# Autodesk Inventor assembly: 4150RobotComplete v3 11.18.14
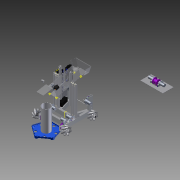
[picture p0: Inventor's stored thumbnail of the model, 180x180]
Saved by Autodesk Inventor 2015 SP1 (Build 190203100, 203)
## iProperties
Created: 2014-09-14
Part Number: 4150RobotComplete v3 11.18.14
Document SubType Name: Assembly
Designer: Family Room
Author: Family Room
## Documents named in this file (35)
- C:\Users\sapatel\Documents\GitHub\CAD\2014_robotComplete\4150RobotComplete v3 11.18.14.iam
- C:\Users\sapatel\Documents\GitHub\CAD\2014_robotComplete\Frame Side.ipt
- C:\Users\sapatel\Documents\GitHub\CAD\2014_robotComplete\center brace.ipt
- C:\Users\sapatel\Documents\GitHub\CAD\2014_robotComplete\Goal Guide 2.ipt
- C:\Users\sapatel\Documents\GitHub\CAD\2014_robotComplete\Hex bearing.ipt
- C:\Users\sapatel\Documents\GitHub\CAD\2014_robotComplete\Axle.ipt
- C:\Users\sapatel\Documents\GitHub\CAD\2014_robotComplete\Hex Collar.ipt
- C:\Users\sapatel\Documents\GitHub\CAD\2014_robotComplete\Hex Sprocket.ipt
- C:\Users\sapatel\Documents\GitHub\CAD\2014_robotComplete\left mecanum.iam
- C:\Users\sapatel\Documents\GitHub\CAD\2014_robotComplete\right mecanum.iam
- C:\Users\sapatel\Documents\GitHub\CAD\2014_robotComplete\Imported Components\motor mount\motor mount.ipt
- C:\Users\sapatel\Documents\GitHub\CAD\2014_robotComplete\Imported Components\motor\motor.iam
- C:\Users\sapatel\Documents\GitHub\CAD\2014_robotComplete\Imported Components\16t Sprocket\16t Sprocket.ipt
- C:\Users\sapatel\Documents\GitHub\CAD\2014_robotComplete\Imported Components\Motor Hub\Motor Hub.ipt
- C:\Users\sapatel\Documents\GitHub\CAD\2014_robotComplete\ball shoot.ipt
- C:\Users\sapatel\Documents\GitHub\CAD\2014_robotComplete\Imported Components\gusset\gusset.ipt
- C:\Users\sapatel\Documents\GitHub\CAD\2014_robotComplete\Lift Section.ipt
- C:\Users\sapatel\Documents\GitHub\CAD\2014_robotComplete\Lift Slider.ipt
- C:\Users\sapatel\Documents\GitHub\CAD\2014_robotComplete\Ball Collection Mechanism.iam
- C:\Users\sapatel\Documents\GitHub\CAD\2014_robotComplete\Bushing .ipt
- C:\Users\sapatel\Documents\GitHub\CAD\2014_robotComplete\BallShoot Axle.ipt
- C:\Users\sapatel\Documents\GitHub\CAD\2014_robotComplete\Rolling_Goal-30cm.iam
- C:\Users\sapatel\Documents\GitHub\CAD\2014_robotComplete\Spinner brace.ipt
- C:\Users\sapatel\Documents\GitHub\CAD\2014_robotComplete\Bushing 1.ipt
- C:\Users\sapatel\Documents\GitHub\CAD\2014_robotComplete\Imported Components\tetrix axle\tetrix axle.ipt
- C:\Users\sapatel\Documents\GitHub\CAD\winch assembly.iam
- C:\Users\sapatel\Documents\GitHub\CAD\2014_robotComplete\Winch baseplate.ipt
- C:\Users\sapatel\Documents\GitHub\CAD\2014_robotComplete\plate 1.ipt
- C:\Users\sapatel\Documents\GitHub\CAD\COTSParts\Tetrix\NXT brick.ipt
- C:\Users\sapatel\Documents\GitHub\CAD\COTSParts\Tetrix\NXT battery cover.ipt
- C:\Users\sapatel\Documents\GitHub\CAD\COTSParts\Tetrix\Tetrix Battery.ipt
- C:\Users\sapatel\Documents\GitHub\CAD\COTSParts\Tetrix\Tetrix DC motor controller.ipt
- C:\Users\sapatel\Documents\GitHub\CAD\COTSParts\Tetrix\Tetrix servo controller.ipt
- C:\Users\sapatel\Documents\GitHub\CAD\COTSParts\Tetrix\Tetrix power switch.ipt
- C:\Users\sapatel\Documents\GitHub\CAD\Electrical\samantha.ipt
## Components (100 placed, 34 different names)
1. Frame Side:2 — Flush:3, Flush:4, Mate:5, Flush:17, Mate:6, Flush:18, Flush:23, Flush:24, Mate:13, Flush:25, Insert:3, Insert:4, Flush:29, Flush:30, Flush:33, Mate:67, Mate:70, Mate:71, Flush:70, Mate:134, Flush:91, Mate:138, Mate:144, Flush:98, Mate:146, Flush:100, Flush:101
2. Frame Side:3 — Flush:3, Flush:4, Mate:7, Mate:15, Flush:26, Insert:1, Insert:2, Flush:27, Flush:28, Mate:63, Flush:31, Mate:65, Mate:72, Flush:71, Mate:132, Mate:142, Flush:97, Mate:147, Flush:102, Flush:103
3. center brace:1 — Mate:6, Flush:18, Mate:7, Flush:24, Mate:14, Mate:16, Angle:2, Angle:3
4. center brace:2 — Mate:5, Flush:17, Flush:23, Mate:90, Mate:117, Flush:96, Mate:143, Mate:145, Flush:99, Flush:107
5. Goal Guide 2:1 — Mate:13, Flush:25, Mate:14
6. Goal Guide 2:2 — Mate:15, Flush:26, Mate:16
7. Hex bearing:1 — Insert:1, Mate:17, Mate:28, Mate:35
8. Hex bearing:2 — Insert:2, Mate:18, Mate:22, Mate:36
9. Hex bearing:3 — Insert:4, Mate:19, Mate:24, Mate:37
10. Hex bearing:4 — Insert:3, Mate:20, Mate:30, Mate:38
11. Axle:1 — Mate:17, Flush:27, Mate:27, Mate:34, Mate:41, Mate:51, Mate:55
12. Axle:2 — Mate:18, Flush:28, Mate:21, Mate:33, Mate:42, Mate:52, Mate:56
13. Axle:3 — Mate:19, Flush:29, Mate:23, Mate:32, Mate:39, Mate:44
14. Axle:4 — Mate:20, Flush:30, Mate:29, Mate:31, Mate:40, Mate:43, Mate:57
15. Hex Collar:1 — Mate:21, Mate:22
16. Hex Collar:2 — Mate:23, Mate:24
17. Hex Collar:3 — Mate:29, Mate:30
18. Hex Collar:4 — Mate:27, Mate:28
19. Hex Sprocket:1 — Mate:31, Mate:38, Mate:46, Flush:41
20. Hex Sprocket:2 — Mate:32, Mate:37, Mate:45
21. Hex Sprocket:3 — Mate:34, Mate:35, Mate:48
22. Hex Sprocket:4 — Mate:33, Mate:36, Mate:47, Flush:39
23. left mecanum:1 [sub-assembly] — Mate:40, Mate:49, Mate:59
24. left mecanum:2 [sub-assembly] — Mate:39, Mate:50, Mate:58, Mate:60
25. Hex Collar:5 — Mate:43, Mate:46, Mate:49
26. Hex Collar:6 — Mate:41, Mate:48, Mate:53
27. Hex Collar:7 — Mate:42, Mate:47, Mate:54
28. Hex Collar:8 — Mate:44, Mate:45, Mate:50
29. right mecanum:1 [sub-assembly] — Mate:52, Mate:54, Mate:61
30. right mecanum:2 [sub-assembly] — Mate:51, Mate:53, Mate:62
31. Hex Collar:9 — Mate:57, Mate:59
32. Hex Collar:10 — Mate:58, Mate:60
33. Hex Collar:11 — Mate:55, Mate:62
34. Hex Collar:12 — Mate:56, Mate:61
35. motor mount:1 — Mate:69, Flush:34, Mate:70, Mate:75, Flush:38
36. motor mount:2 — Flush:33, Mate:67, Mate:69, Flush:34, Mate:71, Mate:76, Flush:37
37. motor mount:3 — Mate:63, Flush:31, Mate:66, Flush:32, Mate:72, Mate:73, Flush:35
38. motor mount:4 — Mate:65, Mate:66, Flush:32, Mate:74, Flush:36
39. motor:1 [sub-assembly] — Mate:73, Flush:35, Mate:80
40. motor:2 [sub-assembly] — Mate:74, Flush:36, Mate:81
41. motor:3 [sub-assembly] — Mate:76, Flush:37, Mate:77
42. motor:4 [sub-assembly] — Mate:75, Flush:38, Mate:78
43. 16t Sprocket:1 — Insert:8, Mate:78, Flush:42
44. 16t Sprocket:2 — Insert:7, Mate:77, Flush:41, Flush:42
45. 16t Sprocket:3 — Insert:9, Flush:39, Flush:40
46. 16t Sprocket:4 — Insert:5, Mate:80, Flush:40
47. Motor Hub:1 — Insert:8
48. Motor Hub:2 — Insert:7
49. Motor Hub:3 — Mate:81, Insert:9
50. Motor Hub:4 — Insert:5
51. ball shoot:1 — Mate:142, Flush:97, Mate:143
52. ball shoot:2 — Mate:144, Flush:98, Mate:145, Mate:158
53. Lift Section:1 — Mate:92, Flush:51, Flush:52, Mate:98, Flush:57, Flush:58, Flush:93, Flush:95, Insert:11
54. Lift Section:2 — Mate:90, Mate:117, Flush:71, Mate:123, Flush:82, Mate:124, Flush:83, Mate:125, Flush:84, Mate:131, Mate:133
55. Lift Slider:1 — Mate:92, Flush:51, Flush:52, Mate:103
56. Lift Slider:3 — Mate:95, Flush:54, Flush:55, Mate:100, Mate:102
57. Lift Slider:4 — Mate:96, Mate:97, Flush:56, Mate:98, Mate:103
58. Lift Section:3 — Mate:95, Flush:54, Flush:55, Flush:59, Flush:60, Mate:111, Flush:66, Mate:112, Flush:69, Angle:1
59. Lift Section:4 — Mate:96, Mate:97, Flush:56, Flush:57, Flush:58, Mate:100, Flush:59, Flush:60, Mate:101, Flush:61, Flush:62
60. Lift Section:5 — Mate:113, Flush:67, Flush:68, Flush:69, Angle:1, Mate:114, Flush:70, Flush:91, Mate:137, Mate:138, Flush:92, Mate:156, Flush:109
61. Lift Section:6 — Mate:118, Flush:72, Flush:73, Mate:121, Flush:78, Flush:79, Flush:83, Flush:84, Flush:85, Flush:86, Mate:127
62. Lift Section:7 — Mate:119, Flush:74, Flush:75, Mate:122, Flush:80, Flush:81, Flush:85, Flush:86, Mate:129, Flush:87, Flush:88
63. Lift Section:8 — Mate:120, Flush:76, Flush:77, Flush:87, Flush:88, Flush:93, Flush:95, Mate:139, Insert:10, Angle:4
64. Lift Slider:5 — Mate:101, Flush:61, Flush:62, Mate:102
65. Lift Slider:6 — Mate:111, Flush:66, Mate:112, Mate:114, Mate:115
66. Lift Slider:7 — Mate:113, Flush:67, Flush:68, Mate:115
67. Lift Slider:8 — Mate:118, Flush:72, Flush:73, Mate:125, Mate:126
68. Lift Slider:9 — Mate:119, Flush:74, Flush:75, Mate:127, Mate:128
69. Lift Slider:10 — Mate:120, Flush:76, Flush:77, Mate:129, Mate:130
70. Lift Slider:11 — Mate:121, Flush:78, Flush:79, Mate:128
71. Lift Slider:12 — Mate:122, Flush:80, Flush:81, Mate:130
72. Lift Slider:13 — Mate:123, Flush:82, Mate:124, Mate:126
73. gusset:1 — Mate:134, Mate:137, Flush:92
74. gusset:2 — Mate:131, Mate:132, Mate:133
75. Ball Collection Mechanism:1 [sub-assembly] — Mate:139, Angle:4, Flush:108
76. Bushing :1 — Insert:10
77. Bushing :2 — Insert:11, Mate:140
78. BallShoot Axle:1 — Mate:140, Flush:96
79. Rolling_Goal-30cm:1 [sub-assembly] — Angle:2, Angle:3
80. Spinner brace:1 — Mate:147, Flush:102, Flush:103, Mate:148, Flush:104, Mate:149, Insert:13
81. Spinner brace:2 — Mate:146, Flush:100, Flush:101, Insert:12, Flush:106
82. motor mount:5 — Mate:148, Flush:104, Mate:149, Mate:150, Flush:105
83. motor:5 [sub-assembly] — Mate:150, Flush:105
84. Bushing 1:1 — Insert:12
85. Bushing 1:2 — Insert:13, Mate:151
86. tetrix axle:1 — Mate:151, Flush:106
87. winch assembly:1 [sub-assembly] — Mate:153, Mate:154, Mate:155
88. Winch baseplate:1 — Mate:153, Mate:154, Mate:155
89. plate 1:1 — Mate:156, Flush:109, Mate:159, Flush:112, Flush:113, Mate:160, Flush:114, Mate:162, Flush:115, Flush:116, Mate:163, Mate:165, Mate:167, Flush:119, Flush:120, Mate:173, Mate:174, Flush:121
90. NXT brick:1 — Mate:157, Flush:110, Flush:111, Flush:119, Flush:120
91. NXT battery cover:1 — Mate:157, Flush:110, Flush:111, Mate:167
92. Tetrix Battery:1 — Mate:158
93. Tetrix DC motor controller:1 — Mate:159, Flush:112, Flush:113, Mate:161
94. Tetrix DC motor controller:2 — Mate:163, Mate:164, Flush:117, Mate:166, Flush:118
95. Tetrix DC motor controller:3 — Mate:162, Flush:115, Flush:116, Mate:164, Flush:117, Flush:122
96. Tetrix servo controller:1 — Mate:160, Mate:161, Flush:114
97. Tetrix DC motor controller:4 — Mate:165, Mate:166, Flush:118
98. Tetrix power switch:1
99. samantha:2 — Mate:173, Mate:174, Flush:121, Flush:122
100. Rolling_Goal-30cm:2 [sub-assembly]
## Relationships (236: Mate 131, Flush 89, Insert 12, Angle 4)
- Flush:3: Frame Side:2 ↔ Frame Side:3
- Flush:4: Frame Side:2 ↔ Frame Side:3
- Mate:5: Frame Side:2 ↔ center brace:2
- Flush:17: Frame Side:2 ↔ center brace:2
- Mate:6: Frame Side:2 ↔ center brace:1
- Flush:18: Frame Side:2 ↔ center brace:1
- Mate:7: Frame Side:3 ↔ center brace:1
- Flush:23 (203.2 mm): Frame Side:2 ↔ center brace:2
- Flush:24 (76.2 mm): Frame Side:2 ↔ center brace:1
- Mate:13: Frame Side:2 ↔ Goal Guide 2:1
- Flush:25: Frame Side:2 ↔ Goal Guide 2:1
- Mate:14: center brace:1 ↔ Goal Guide 2:1
- Mate:15: Frame Side:3 ↔ Goal Guide 2:2
- Flush:26: Frame Side:3 ↔ Goal Guide 2:2
- Mate:16: center brace:1 ↔ Goal Guide 2:2
- Insert:1: Frame Side:3 ↔ Hex bearing:1
- Insert:2: Frame Side:3 ↔ Hex bearing:2
- Insert:3: Frame Side:2 ↔ Hex bearing:4
- Insert:4: Frame Side:2 ↔ Hex bearing:3
- Mate:17: Hex bearing:1 ↔ Axle:1
- Flush:27: Frame Side:3 ↔ Axle:1
- Mate:18: Hex bearing:2 ↔ Axle:2
- Flush:28: Frame Side:3 ↔ Axle:2
- Mate:19: Hex bearing:3 ↔ Axle:3
- Mate:20: Hex bearing:4 ↔ Axle:4
- Flush:29: Frame Side:2 ↔ Axle:3
- Flush:30: Frame Side:2 ↔ Axle:4
- Mate:21: Axle:2 ↔ Hex Collar:1
- Mate:22: Hex bearing:2 ↔ Hex Collar:1
- Mate:23: Axle:3 ↔ Hex Collar:2
- Mate:24: Hex bearing:3 ↔ Hex Collar:2
- Mate:27: Axle:1 ↔ Hex Collar:4
- Mate:28: Hex bearing:1 ↔ Hex Collar:4
- Mate:29: Axle:4 ↔ Hex Collar:3
- Mate:30: Hex bearing:4 ↔ Hex Collar:3
- Mate:31: Axle:4 ↔ Hex Sprocket:1
- Mate:32: Axle:3 ↔ Hex Sprocket:2
- Mate:33: Axle:2 ↔ Hex Sprocket:4
- Mate:34: Axle:1 ↔ Hex Sprocket:3
- Mate:35: Hex bearing:1 ↔ Hex Sprocket:3
- Mate:36: Hex bearing:2 ↔ Hex Sprocket:4
- Mate:37: Hex bearing:3 ↔ Hex Sprocket:2
- Mate:38: Hex bearing:4 ↔ Hex Sprocket:1
- Mate:39: Axle:3 ↔ left mecanum:2
- Mate:40: Axle:4 ↔ left mecanum:1
- Mate:41: Axle:1 ↔ Hex Collar:6
- Mate:42: Axle:2 ↔ Hex Collar:7
- Mate:43: Axle:4 ↔ Hex Collar:5
- Mate:44: Axle:3 ↔ Hex Collar:8
- Mate:45: Hex Sprocket:2 ↔ Hex Collar:8
- Mate:46: Hex Sprocket:1 ↔ Hex Collar:5
- Mate:47: Hex Sprocket:4 ↔ Hex Collar:7
- Mate:48: Hex Sprocket:3 ↔ Hex Collar:6
- Mate:49: left mecanum:1 ↔ Hex Collar:5
- Mate:50: left mecanum:2 ↔ Hex Collar:8
- Mate:51: Axle:1 ↔ right mecanum:2
- Mate:52: Axle:2 ↔ right mecanum:1
- Mate:53: Hex Collar:6 ↔ right mecanum:2
- Mate:54: Hex Collar:7 ↔ right mecanum:1
- Mate:55: Axle:1 ↔ Hex Collar:11
- Mate:56: Axle:2 ↔ Hex Collar:12
- Mate:57: Axle:4 ↔ Hex Collar:9
- Mate:58: left mecanum:2 ↔ Hex Collar:10
- Mate:59: left mecanum:1 ↔ Hex Collar:9
- Mate:60: left mecanum:2 ↔ Hex Collar:10
- Mate:61: right mecanum:1 ↔ Hex Collar:12
- Mate:62: right mecanum:2 ↔ Hex Collar:11
- Mate:63: Frame Side:3 ↔ motor mount:3
- Flush:31: Frame Side:3 ↔ motor mount:3
- Mate:65: Frame Side:3 ↔ motor mount:4
- Mate:66: motor mount:3 ↔ motor mount:4
- Flush:32: motor mount:3 ↔ motor mount:4
- Flush:33: Frame Side:2 ↔ motor mount:2
- Mate:67: Frame Side:2 ↔ motor mount:2
- Mate:69: motor mount:1 ↔ motor mount:2
- Flush:34: motor mount:1 ↔ motor mount:2
- Mate:70: Frame Side:2 ↔ motor mount:1
- Mate:71: Frame Side:2 ↔ motor mount:2
- Mate:72: Frame Side:3 ↔ motor mount:3
- Mate:73: motor mount:3 ↔ motor:1
- Mate:74: motor mount:4 ↔ motor:2
- Mate:75: motor mount:1 ↔ motor:4
- Mate:76: motor mount:2 ↔ motor:3
- Flush:35: motor mount:3 ↔ motor:1
- Flush:36: motor mount:4 ↔ motor:2
- Flush:37: motor mount:2 ↔ motor:3
- Flush:38: motor mount:1 ↔ motor:4
- Insert:5: 16t Sprocket:4 ↔ Motor Hub:4
- Insert:7: 16t Sprocket:2 ↔ Motor Hub:2
- Insert:8: 16t Sprocket:1 ↔ Motor Hub:1
- Mate:77: motor:3 ↔ 16t Sprocket:2
- Mate:78: motor:4 ↔ 16t Sprocket:1
- Mate:80: motor:1 ↔ 16t Sprocket:4
- Mate:81: motor:2 ↔ Motor Hub:3
- Insert:9: 16t Sprocket:3 ↔ Motor Hub:3
- Flush:39: Hex Sprocket:4 ↔ 16t Sprocket:3
- Flush:40: 16t Sprocket:3 ↔ 16t Sprocket:4
- Flush:41: Hex Sprocket:1 ↔ 16t Sprocket:2
- Flush:42: 16t Sprocket:1 ↔ 16t Sprocket:2
- Mate:90: center brace:2 ↔ Lift Section:2
- Mate:92: Lift Section:1 ↔ Lift Slider:1
- Flush:51: Lift Section:1 ↔ Lift Slider:1
- Flush:52: Lift Section:1 ↔ Lift Slider:1
- Mate:95: Lift Slider:3 ↔ Lift Section:3
- Flush:54: Lift Slider:3 ↔ Lift Section:3
- Flush:55: Lift Slider:3 ↔ Lift Section:3
- Mate:96: Lift Slider:4 ↔ Lift Section:4
- Mate:97: Lift Slider:4 ↔ Lift Section:4
- Flush:56: Lift Slider:4 ↔ Lift Section:4
- Mate:98: Lift Section:1 ↔ Lift Slider:4
- Flush:57: Lift Section:1 ↔ Lift Section:4
- Flush:58: Lift Section:1 ↔ Lift Section:4
- Mate:100: Lift Slider:3 ↔ Lift Section:4
- Flush:59: Lift Section:3 ↔ Lift Section:4
- Flush:60: Lift Section:3 ↔ Lift Section:4
- Mate:101: Lift Section:4 ↔ Lift Slider:5
- Flush:61: Lift Section:4 ↔ Lift Slider:5
- Flush:62: Lift Section:4 ↔ Lift Slider:5
- Mate:102: Lift Slider:3 ↔ Lift Slider:5
- Mate:103: Lift Slider:1 ↔ Lift Slider:4
- Mate:111: Lift Section:3 ↔ Lift Slider:6
- Flush:66: Lift Section:3 ↔ Lift Slider:6
- Mate:112: Lift Section:3 ↔ Lift Slider:6
- Mate:113: Lift Section:5 ↔ Lift Slider:7
- Flush:67: Lift Section:5 ↔ Lift Slider:7
- Flush:68: Lift Section:5 ↔ Lift Slider:7
- Flush:69: Lift Section:3 ↔ Lift Section:5
- Angle:1 (0 deg): Lift Section:3 ↔ Lift Section:5
- Mate:114: Lift Section:5 ↔ Lift Slider:6
- Mate:115: Lift Slider:6 ↔ Lift Slider:7
- Flush:70: Frame Side:2 ↔ Lift Section:5
- Mate:117: center brace:2 ↔ Lift Section:2
- Flush:71: Frame Side:3 ↔ Lift Section:2
- Mate:118: Lift Section:6 ↔ Lift Slider:8
- Flush:72: Lift Section:6 ↔ Lift Slider:8
- Flush:73: Lift Section:6 ↔ Lift Slider:8
- Mate:119: Lift Section:7 ↔ Lift Slider:9
- Flush:74: Lift Section:7 ↔ Lift Slider:9
- Flush:75: Lift Section:7 ↔ Lift Slider:9
- Mate:120: Lift Section:8 ↔ Lift Slider:10
- Flush:76: Lift Section:8 ↔ Lift Slider:10
- Flush:77: Lift Section:8 ↔ Lift Slider:10
- Mate:121: Lift Section:6 ↔ Lift Slider:11
- Flush:78: Lift Section:6 ↔ Lift Slider:11
- Flush:79: Lift Section:6 ↔ Lift Slider:11
- Mate:122: Lift Section:7 ↔ Lift Slider:12
- Flush:80: Lift Section:7 ↔ Lift Slider:12
- Flush:81: Lift Section:7 ↔ Lift Slider:12
- Mate:123: Lift Section:2 ↔ Lift Slider:13
- Flush:82: Lift Section:2 ↔ Lift Slider:13
- Mate:124: Lift Section:2 ↔ Lift Slider:13
- Flush:83: Lift Section:2 ↔ Lift Section:6
- Mate:125: Lift Section:2 ↔ Lift Slider:8
- Flush:84: Lift Section:2 ↔ Lift Section:6
- Mate:126: Lift Slider:8 ↔ Lift Slider:13
- Flush:85: Lift Section:6 ↔ Lift Section:7
- Flush:86: Lift Section:6 ↔ Lift Section:7
- Mate:127: Lift Section:6 ↔ Lift Slider:9
- Mate:128: Lift Slider:9 ↔ Lift Slider:11
- Mate:129: Lift Section:7 ↔ Lift Slider:10
- Flush:87: Lift Section:7 ↔ Lift Section:8
- Flush:88: Lift Section:7 ↔ Lift Section:8
- Mate:130: Lift Slider:10 ↔ Lift Slider:12
- Mate:131: Lift Section:2 ↔ gusset:2
- Mate:132: Frame Side:3 ↔ gusset:2
- Mate:133: Lift Section:2 ↔ gusset:2
- Mate:134: Frame Side:2 ↔ gusset:1
- Flush:91: Frame Side:2 ↔ Lift Section:5
- Mate:137: Lift Section:5 ↔ gusset:1
- Mate:138: Frame Side:2 ↔ Lift Section:5
- Flush:92: Lift Section:5 ↔ gusset:1
- Flush:93: Lift Section:1 ↔ Lift Section:8
- Flush:95: Lift Section:1 ↔ Lift Section:8
- Mate:139: Lift Section:8 ↔ Ball Collection Mechanism:1
- Insert:10: Lift Section:8 ↔ Bushing :1
- Insert:11: Lift Section:1 ↔ Bushing :2
- Mate:140: Bushing :2 ↔ BallShoot Axle:1
- Flush:96: center brace:2 ↔ BallShoot Axle:1
- Angle:2 (0 deg): center brace:1 ↔ Rolling_Goal-30cm:1
- Angle:3 (0 deg): center brace:1 ↔ Rolling_Goal-30cm:1
- Mate:142: Frame Side:3 ↔ ball shoot:1
- Flush:97: Frame Side:3 ↔ ball shoot:1
- Mate:143: center brace:2 ↔ ball shoot:1
- Mate:144: Frame Side:2 ↔ ball shoot:2
- Flush:98: Frame Side:2 ↔ ball shoot:2
- Mate:145: center brace:2 ↔ ball shoot:2
- Flush:99: center brace:2
- Angle:4 (165 deg): Lift Section:8 ↔ Ball Collection Mechanism:1
- Mate:146: Frame Side:2 ↔ Spinner brace:2
- Flush:100: Frame Side:2 ↔ Spinner brace:2
- Flush:101: Frame Side:2 ↔ Spinner brace:2
- Mate:147: Frame Side:3 ↔ Spinner brace:1
- Flush:102: Frame Side:3 ↔ Spinner brace:1
- Flush:103: Frame Side:3 ↔ Spinner brace:1
- Mate:148: Spinner brace:1 ↔ motor mount:5
- Flush:104: Spinner brace:1 ↔ motor mount:5
- Mate:149: Spinner brace:1 ↔ motor mount:5
- Mate:150: motor mount:5 ↔ motor:5
- Flush:105: motor mount:5 ↔ motor:5
- Insert:12: Spinner brace:2 ↔ Bushing 1:1
- Insert:13: Spinner brace:1 ↔ Bushing 1:2
- Mate:151: Bushing 1:2 ↔ tetrix axle:1
- Flush:106 (25.4 mm): Spinner brace:2 ↔ tetrix axle:1
- Mate:153: winch assembly:1 ↔ Winch baseplate:1
- Mate:154: winch assembly:1 ↔ Winch baseplate:1
- Mate:155: winch assembly:1 ↔ Winch baseplate:1
- Flush:107: center brace:2
- Flush:108: Ball Collection Mechanism:1
- Mate:156: Lift Section:5 ↔ plate 1:1
- Flush:109: Lift Section:5 ↔ plate 1:1
- Mate:157: NXT brick:1 ↔ NXT battery cover:1
- Flush:110 (-60.9854 mm): NXT brick:1 ↔ NXT battery cover:1
- Flush:111: NXT brick:1 ↔ NXT battery cover:1
- Mate:158: ball shoot:2 ↔ Tetrix Battery:1
- Mate:159: plate 1:1 ↔ Tetrix DC motor controller:1
- Flush:112: plate 1:1 ↔ Tetrix DC motor controller:1
- Flush:113 (10.16 mm): plate 1:1 ↔ Tetrix DC motor controller:1
- Mate:160: plate 1:1 ↔ Tetrix servo controller:1
- Mate:161: Tetrix DC motor controller:1 ↔ Tetrix servo controller:1
- Flush:114 (10.16 mm): plate 1:1 ↔ Tetrix servo controller:1
- Mate:162: plate 1:1 ↔ Tetrix DC motor controller:3
- Flush:115: plate 1:1 ↔ Tetrix DC motor controller:3
- Flush:116 (35.814 mm): plate 1:1 ↔ Tetrix DC motor controller:3
- Mate:163: plate 1:1 ↔ Tetrix DC motor controller:2
- Mate:164: Tetrix DC motor controller:2 ↔ Tetrix DC motor controller:3
- Flush:117: Tetrix DC motor controller:2 ↔ Tetrix DC motor controller:3
- Mate:165: plate 1:1 ↔ Tetrix DC motor controller:4
- Mate:166: Tetrix DC motor controller:2 ↔ Tetrix DC motor controller:4
- Flush:118: Tetrix DC motor controller:2 ↔ Tetrix DC motor controller:4
- Mate:167: plate 1:1 ↔ NXT battery cover:1
- Flush:119 (76.2 mm): plate 1:1 ↔ NXT brick:1
- Flush:120: plate 1:1 ↔ NXT brick:1
- Mate:173: plate 1:1 ↔ samantha:2
- Mate:174: plate 1:1 ↔ samantha:2
- Flush:121 (8.5598 mm): plate 1:1 ↔ samantha:2
- Flush:122: Tetrix DC motor controller:3 ↔ samantha:2
